# Autodesk Inventor assembly: 4830902 DPDM-6-15-PA---(0)
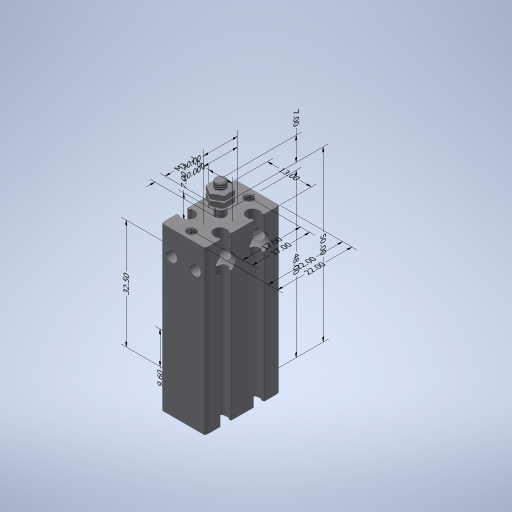
[picture p0: Inventor's stored thumbnail of the model, 512x512]
Saved by Autodesk Inventor 2024.1 (Build 281209000, 209)
## iProperties
Created: 2024-05-27
Part Number: 4830902 DPDM-6-15-PA---(0)
Catalog Web Link: www.cadenas.de
Description: DPDM-compact cylinder
Vendor: FESTO
Document SubType Name: Assembly
Designer: psAdmin
Manufacturer: FESTO
Mass: 30.15 g
Surface Area: 69.305 cm^2
Volume: 10.4892 cm^3
Density: 2.87439 g/cm^3
Category: PARTsolutions
Company: FESTO
PSOL_IDENT_0: {ATYP=ASSISTANT},{DATA=script=$CADENAS_DATA/23d-libs/festo/webfesto.vbb&M_FAMILY=DPDM&M_GROUP=01&M_P
PSOL_IDENT_1: ARTNO=4830902&IDCODE1=DPDM-6-15-PA&IDCODE2=&customer_number_cns=&MATES=1&LOD=HI&LOCKERP=0&SINGLEPART=
PSOL_IDENT_2: 1}
NB: 4830902 DPDM-6-15-PA---(0)
NN: DPDM
NT: compact cylinder
NBSYN: $TNR. $TYP.$VERNB.-$KOL.-$HUB.$FUNNB.$KOTNB.-$DAEM.$POS.$TEMNB.$BWENB.---($HUBST.)
LINA: 4830902 DPDM-6-15-PA
CATALOG: Festo
TNR: 4830902
TYP: DPDM
VER: -
KOL: 6
HUB: 15
HUBST: 0
FUN: -
KOT: -
DAEM: P
POS: A
TEM: -
BWE: -
AM: 7
KK: M3
WH: 2
MM: 3
SW: 0
LS: 0
ZJ: 35
L2: 33
EE: M5
ET: 4
BG: 5
RT: M3
H2: 10
E: 13
UO: 22
TO: 17
H3: 7
LX: 7
PL: 17.5
PR: 9.5
U1: 0
D5: 3.3
D6: 6
T1: 5
B3: 11
H4: 10.5
H5: 17.5
L4: 42
L5: 9
L6: 0
ZM: 37
L8: 44
D8: 0
W22: 0
H7: 5.5
H8: 1.8
CNSMASSEXACT: 0.03
GTIN: 4052568292546
SUPPLIER: FESTO
ARTICLENO: 4830902 DPDM-6-15-PA---(0)
BOMINFO: 4830902 DPDM-6-15-PA
CREATOR: CADENAS GmbH
Title: 4830902 DPDM-6-15-PA
Author: Cadenas PARTsolutions
Comments: compact cylinder
## Documents named in this file (4)
- C:\Users\Krzysiu\Documents\Inventor\4830902 DPDM-6-15-PA---(0).iam
- C:\Users\Krzysiu\Documents\Inventor\4674228 DPDM-15---(h).ipt
- C:\Users\Krzysiu\Documents\Inventor\4674228 DPDM-15---(r).ipt
- C:\Users\Krzysiu\Documents\Inventor\ISO 4035 M3(F).ipt
## Components (4 placed, 3 different names)
1. 4674228 DPDM-15---(h):1 — CP_ROD1_XY@1 <-> CP1_XY@2, CP_ROD1_Z@1 <-> CP1_Z@2, CP_ROD1_YZ@1 <-> CP1_YZ@2
2. 4674228 DPDM-15---(r):1 — CP_ROD1_XY@1 <-> CP1_XY@2, CP_ROD1_Z@1 <-> CP1_Z@2, CP_ROD1_YZ@1 <-> CP1_YZ@2, NUT_CP_6_10_1_XY@2 <-> IP2_XY@3, NUT_CP_6_10_1_Z@2 <-> IP2_Z@3, NUT_CP_6_10_1_YZ@2 <-> IP2_YZ@3, NUT_CP_6_10_2_XY@2 <-> IP2_XY@4, NUT_CP_6_10_2_Z@2 <-> IP2_Z@4, NUT_CP_6_10_2_YZ@2 <-> IP2_YZ@4
3. ISO 4035 M3(F):1 — NUT_CP_6_10_1_XY@2 <-> IP2_XY@3, NUT_CP_6_10_1_Z@2 <-> IP2_Z@3, NUT_CP_6_10_1_YZ@2 <-> IP2_YZ@3
4. ISO 4035 M3(F):2 — NUT_CP_6_10_2_XY@2 <-> IP2_XY@4, NUT_CP_6_10_2_Z@2 <-> IP2_Z@4, NUT_CP_6_10_2_YZ@2 <-> IP2_YZ@4
## Relationships (9: Mate 4, Angle 3, Flush 2)
- CP_ROD1_XY@1 <-> CP1_XY@2 [Mate]: 4674228 DPDM-15---(h):1 ↔ 4674228 DPDM-15---(r):1
- CP_ROD1_Z@1 <-> CP1_Z@2 [Mate]: 4674228 DPDM-15---(h):1 ↔ 4674228 DPDM-15---(r):1
- CP_ROD1_YZ@1 <-> CP1_YZ@2 [Angle] (0 deg): 4674228 DPDM-15---(h):1 ↔ 4674228 DPDM-15---(r):1
- NUT_CP_6_10_1_XY@2 <-> IP2_XY@3 [Flush]: 4674228 DPDM-15---(r):1 ↔ ISO 4035 M3(F):1
- NUT_CP_6_10_1_Z@2 <-> IP2_Z@3 [Mate]: 4674228 DPDM-15---(r):1 ↔ ISO 4035 M3(F):1
- NUT_CP_6_10_1_YZ@2 <-> IP2_YZ@3 [Angle] (0 deg): 4674228 DPDM-15---(r):1 ↔ ISO 4035 M3(F):1
- NUT_CP_6_10_2_XY@2 <-> IP2_XY@4 [Flush]: 4674228 DPDM-15---(r):1 ↔ ISO 4035 M3(F):2
- NUT_CP_6_10_2_Z@2 <-> IP2_Z@4 [Mate]: 4674228 DPDM-15---(r):1 ↔ ISO 4035 M3(F):2
- NUT_CP_6_10_2_YZ@2 <-> IP2_YZ@4 [Angle] (0 deg): 4674228 DPDM-15---(r):1 ↔ ISO 4035 M3(F):2
